# Autodesk Inventor assembly: tower 3
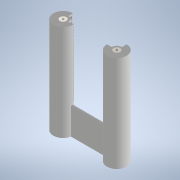
[picture p0: Inventor's stored thumbnail of the model, 180x180]
Saved by Autodesk Inventor 2020.1 (Build 241239000, 239)
## iProperties
Created: 2022-04-02
Part Number: tower 3
Document SubType Name: Assembly
Designer: User
Author: User
## Documents named in this file (3)
- D:\GitHub\TANK\3D-turret\tower 3.iam
- D:\GitHub\TANK\3D-turret\gun 3.iam
- D:\GitHub\TANK\3D-turret\gun 3_ЗЕРКАЛО.iam
## Components (2 placed, 2 different names)
1. gun 3:1 [sub-assembly] — Жесткий:1
2. gun 3_ЗЕРКАЛО:1 [sub-assembly] — Жесткий:1
## Relationships (1: WeldJoint 1)
- Жесткий:1 [WeldJoint]: gun 3:1 ↔ gun 3_ЗЕРКАЛО:1
